# Autodesk Inventor assembly: Robot
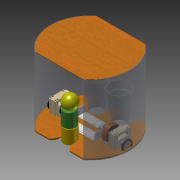
[picture p0: Inventor's stored thumbnail of the model, 180x180]
Saved by Autodesk Inventor 2014 SP1 (Build 180222100, 222)
## iProperties
Created: 2015-03-22
Part Number: Robot
Document SubType Name: Assembly
Designer: david
Mass: 1224.47 g
Surface Area: 3724.37 cm^2
Volume: 783.381 cm^3
Density: 1.56306 g/cm^3
Author: david
## Documents named in this file (19)
- C:\Users\asus\Documents\Autodesk\Projects\AUSBEEDone\Coupe2015\Robot.iam
- C:\Users\asus\Documents\Autodesk\Projects\AUSBEEDone\Components\EncoderBlock.iam
- C:\Users\asus\Documents\Autodesk\Projects\AUSBEEDone\Components\EncoderSupportOutside.ipt
- C:\Users\asus\Documents\Autodesk\Projects\AUSBEEDone\Components\Fasteners\ThreadedRod_M3_EncoderSupportInside.ipt
- C:\Users\asus\Documents\Autodesk\Projects\AUSBEEDone\Components\Fasteners\ThreadedRod_M3_EncoderSupportChassis.ipt
- C:\Users\asus\Documents\Autodesk\Projects\AUSBEEDone\Components\Fasteners\NylstopNut_M3.ipt
- C:\Users\asus\Documents\Autodesk\Projects\AUSBEEDone\Components\Fasteners\CompressionCoilSpring_5.5x35.ipt
- C:\Users\asus\Documents\Autodesk\Projects\AUSBEEDone\Components\Linking\Bracket.ipt
- C:\Users\asus\Documents\Autodesk\Projects\AUSBEEDone\Components\Linking\BracketUnfolded.ipt
- C:\Users\asus\Documents\Autodesk\Projects\AUSBEEDone\Components\Linking\BracketHalf.ipt
- C:\Users\asus\Documents\Autodesk\Projects\AUSBEEDone\Components\Motors\MotorBlockOneWheel.iam
- C:\Users\asus\Documents\Autodesk\Projects\AUSBEEDone\Coupe2015\ChassisRound.ipt
- C:\Users\asus\Documents\Autodesk\Projects\AUSBEEDone\Components\Motors\MotorBlockTwoWheels.iam
- C:\Users\asus\Documents\Autodesk\Projects\AUSBEEDone\Coupe2015\RoofRound.ipt
- C:\Users\asus\Documents\Autodesk\Projects\AUSBEEDone\Coupe2015\SideRound.ipt
- C:\Users\asus\Documents\Autodesk\Projects\AUSBEEDone\Coupe2015\PlayingElements\LightBulb_MaxSize.ipt
- C:\Users\asus\Documents\Autodesk\Projects\AUSBEEDone\Coupe2015\PlayingElements\StandGreen.ipt
- C:\Users\asus\Documents\Autodesk\Projects\AUSBEEDone\Coupe2015\PlayingElements\StandYellow.ipt
- C:\Users\asus\Documents\Autodesk\Projects\AUSBEEDone\Coupe2015\PlayingElements\PopcornCup.ipt
## Components (73 placed, 18 different names)
1. ChassisRound:1 — Mate:1, Mate:2, Cylindrical:25, Cylindrical:26, Mate:15, Mate:16, Mate:17, Mate:18, Mate:28, Mate:29, Mate:30, Mate:31, Mate:97, Mate:98, Angle:1, Mate:106, Mate:107, Angle:2, Mate:121, Mate:122, Mate:123, Mate:124, Mate:125, Mate:126, Mate:127
2. EncoderBlock:1 [sub-assembly] — Cylindrical:5, Cylindrical:6, Cylindrical:7, Cylindrical:8, Mate:7, Mate:8, Mate:9, Mate:10, Mate:44, Mate:45, Mate:46, Mate:47
3. EncoderBlock:2 [sub-assembly] — Cylindrical:9, Cylindrical:10, Cylindrical:11, Cylindrical:12, Mate:3, Mate:4, Mate:5, Mate:6, Flush:16, Mate:38, Mate:39, Mate:40, Tangent:1
4. MotorBlockOneWheel:1 [sub-assembly] — Mate:112, Mate:113, Mate:114
5. MotorBlockTwoWheels:1 [sub-assembly] — Mate:117, Mate:118, Mate:119, Mate:120
6. EncoderSupportOutside:1 — Cylindrical:1, Cylindrical:2, Cylindrical:3, Cylindrical:4, Mate:1, Cylindrical:21, Cylindrical:22, Cylindrical:23, Cylindrical:24, Flush:17
7. EncoderSupportOutside:2 — Mate:2, Cylindrical:13, Cylindrical:14, Cylindrical:15, Cylindrical:16, Cylindrical:29, Cylindrical:30, Cylindrical:31, Cylindrical:32, Mate:37
8. ThreadedRod_M3_EncoderSupportInside:1 — Cylindrical:3, Cylindrical:7, Mate:10, Mate:49, Mate:56, Flush:20
9. ThreadedRod_M3_EncoderSupportInside:2 — Cylindrical:1, Cylindrical:8, Mate:8, Mate:50, Mate:59, Flush:18
10. ThreadedRod_M3_EncoderSupportInside:3 — Cylindrical:4, Cylindrical:6, Mate:7, Mate:51, Mate:58, Flush:19
11. ThreadedRod_M3_EncoderSupportInside:4 — Cylindrical:2, Cylindrical:5, Mate:9, Mate:48, Mate:57, Flush:21
12. ThreadedRod_M3_EncoderSupportInside:5 — Cylindrical:9, Cylindrical:14, Mate:5, Mate:42, Mate:52, Flush:23
13. ThreadedRod_M3_EncoderSupportInside:6 — Cylindrical:10, Cylindrical:16, Mate:4, Mate:41, Mate:53, Flush:22
14. ThreadedRod_M3_EncoderSupportInside:7 — Cylindrical:12, Cylindrical:13, Mate:6, Mate:43, Mate:55, Flush:25
15. ThreadedRod_M3_EncoderSupportInside:8 — Cylindrical:11, Cylindrical:15, Mate:3, Mate:36, Mate:54, Flush:24
16. ThreadedRod_M3_EncoderSupportChassis:1 — Cylindrical:22, Mate:24, Flush:11, Mate:33, Flush:15, Mate:121
17. ThreadedRod_M3_EncoderSupportChassis:2 — Cylindrical:21, Mate:25, Flush:10, Mate:32, Flush:12
18. ThreadedRod_M3_EncoderSupportChassis:3 — Cylindrical:24, Mate:26, Flush:9, Flush:14, Mate:35, Mate:122
19. ThreadedRod_M3_EncoderSupportChassis:4 — Cylindrical:23, Mate:27, Flush:8, Mate:34, Flush:13
20. ThreadedRod_M3_EncoderSupportChassis:5 — Cylindrical:29, Mate:12, Flush:2, Mate:22, Flush:6
21. ThreadedRod_M3_EncoderSupportChassis:6 — Cylindrical:30, Mate:11, Flush:1, Mate:21, Flush:7
22. ThreadedRod_M3_EncoderSupportChassis:7 — Cylindrical:25, Cylindrical:32, Flush:3, Mate:13, Mate:19, Mate:23
23. ThreadedRod_M3_EncoderSupportChassis:8 — Cylindrical:26, Cylindrical:31, Mate:14, Flush:4, Mate:20, Flush:5
24. NylstopNut_M3:1 — Mate:14, Flush:4, Mate:16
25. NylstopNut_M3:2 — Flush:3, Mate:13, Mate:15
26. NylstopNut_M3:3 — Mate:11, Flush:1, Mate:17
27. NylstopNut_M3:4 — Mate:12, Flush:2, Mate:18
28. NylstopNut_M3:5 — Mate:20, Flush:5
29. NylstopNut_M3:6 — Mate:22, Flush:6
30. NylstopNut_M3:7 — Mate:21, Flush:7
31. NylstopNut_M3:8 — Mate:19, Mate:23
32. NylstopNut_M3:9 — Mate:27, Flush:8, Mate:31
33. NylstopNut_M3:10 — Mate:26, Flush:9, Mate:30
34. NylstopNut_M3:11 — Mate:25, Flush:10, Mate:29
35. NylstopNut_M3:12 — Mate:24, Flush:11, Mate:28
36. NylstopNut_M3:13 — Mate:33, Flush:15
37. NylstopNut_M3:14 — Mate:34, Flush:13
38. NylstopNut_M3:15 — Mate:32, Flush:12
39. NylstopNut_M3:16 — Flush:14, Mate:35
40. CompressionCoilSpring_5.5x35:1 — Mate:36, Flush:16, Mate:37
41. CompressionCoilSpring_5.5x35:2 — Mate:40, Mate:41
42. CompressionCoilSpring_5.5x35:3 — Mate:39, Mate:42
43. CompressionCoilSpring_5.5x35:4 — Mate:38, Mate:43
44. CompressionCoilSpring_5.5x35:5 — Mate:44, Mate:48, Flush:17
45. CompressionCoilSpring_5.5x35:6 — Mate:45, Mate:49
46. CompressionCoilSpring_5.5x35:7 — Mate:46, Mate:50
47. CompressionCoilSpring_5.5x35:8 — Mate:47, Mate:51
48. NylstopNut_M3:17 — Mate:57, Flush:21
49. NylstopNut_M3:18 — Mate:56, Flush:20
50. NylstopNut_M3:19 — Mate:59, Flush:18
51. NylstopNut_M3:20 — Mate:58, Flush:19
52. NylstopNut_M3:21 — Mate:52, Flush:23
53. NylstopNut_M3:22 — Mate:53, Flush:22
54. NylstopNut_M3:23 — Mate:55, Flush:25
55. NylstopNut_M3:24 — Mate:54, Flush:24
56. Bracket:1 — Mate:60, Mate:61, Mate:62, Mate:98, Mate:117, Mate:119
57. Bracket:2 — Mate:74, Mate:75, Mate:76, Mate:114
58. BracketUnfolded:1 — Mate:60, Mate:61, Mate:62, Mate:68, Mate:70, Mate:102
59. Bracket:3 — Mate:81, Mate:82, Mate:83, Mate:97, Mate:107, Mate:118, Mate:120
60. Bracket:4 — Mate:84, Mate:85, Mate:86, Mate:106, Mate:112, Mate:113
61. BracketUnfolded:4 — Mate:69, Mate:71, Mate:74, Mate:75, Mate:76, Mate:101
62. BracketHalf:1 — Mate:87, Mate:88, Mate:89, Mate:90, Mate:103
63. BracketHalf:2 — Mate:68, Mate:69, Mate:70, Mate:71, Mate:101, Mate:102
64. BracketUnfolded:5 — Mate:81, Mate:82, Mate:83, Mate:89, Mate:90, Mate:103
65. BracketUnfolded:6 — Mate:84, Mate:85, Mate:86, Mate:87, Mate:88
66. RoofRound:1 — Mate:128, Mate:129, Mate:131
67. SideRound:1 — Mate:125, Mate:126, Mate:127, Mate:128, Mate:129
68. SideRound:2 — Mate:123, Mate:124, Mate:131
69. LightBulb_MaxSize:1
70. StandGreen:1
71. StandYellow:1
72. PopcornCup:2
73. PopcornCup:4
## Relationships (157: Mate 103, CylindricalJoint 26, Flush 25, Angle 2, Tangent 1)
- Cylindrical:1: EncoderSupportOutside:1 ↔ ThreadedRod_M3_EncoderSupportInside:2
- Cylindrical:2: EncoderSupportOutside:1 ↔ ThreadedRod_M3_EncoderSupportInside:4
- Cylindrical:3: EncoderSupportOutside:1 ↔ ThreadedRod_M3_EncoderSupportInside:1
- Cylindrical:4: EncoderSupportOutside:1 ↔ ThreadedRod_M3_EncoderSupportInside:3
- Cylindrical:5: EncoderBlock:1 ↔ ThreadedRod_M3_EncoderSupportInside:4
- Mate:1: ChassisRound:1 ↔ EncoderSupportOutside:1
- Cylindrical:6: EncoderBlock:1 ↔ ThreadedRod_M3_EncoderSupportInside:3
- Cylindrical:7: EncoderBlock:1 ↔ ThreadedRod_M3_EncoderSupportInside:1
- Cylindrical:8: EncoderBlock:1 ↔ ThreadedRod_M3_EncoderSupportInside:2
- Mate:2: ChassisRound:1 ↔ EncoderSupportOutside:2
- Cylindrical:9: EncoderBlock:2 ↔ ThreadedRod_M3_EncoderSupportInside:5
- Cylindrical:10: EncoderBlock:2 ↔ ThreadedRod_M3_EncoderSupportInside:6
- Cylindrical:11: EncoderBlock:2 ↔ ThreadedRod_M3_EncoderSupportInside:8
- Cylindrical:12: EncoderBlock:2 ↔ ThreadedRod_M3_EncoderSupportInside:7
- Cylindrical:13: EncoderSupportOutside:2 ↔ ThreadedRod_M3_EncoderSupportInside:7
- Cylindrical:14: EncoderSupportOutside:2 ↔ ThreadedRod_M3_EncoderSupportInside:5
- Cylindrical:15: EncoderSupportOutside:2 ↔ ThreadedRod_M3_EncoderSupportInside:8
- Cylindrical:16: EncoderSupportOutside:2 ↔ ThreadedRod_M3_EncoderSupportInside:6
- Cylindrical:21: EncoderSupportOutside:1 ↔ ThreadedRod_M3_EncoderSupportChassis:2
- Cylindrical:22: EncoderSupportOutside:1 ↔ ThreadedRod_M3_EncoderSupportChassis:1
- Cylindrical:23: EncoderSupportOutside:1 ↔ ThreadedRod_M3_EncoderSupportChassis:4
- Cylindrical:24: EncoderSupportOutside:1 ↔ ThreadedRod_M3_EncoderSupportChassis:3
- Cylindrical:25: ChassisRound:1 ↔ ThreadedRod_M3_EncoderSupportChassis:7
- Cylindrical:26: ChassisRound:1 ↔ ThreadedRod_M3_EncoderSupportChassis:8
- Cylindrical:29: EncoderSupportOutside:2 ↔ ThreadedRod_M3_EncoderSupportChassis:5
- Cylindrical:30: EncoderSupportOutside:2 ↔ ThreadedRod_M3_EncoderSupportChassis:6
- Cylindrical:31: EncoderSupportOutside:2 ↔ ThreadedRod_M3_EncoderSupportChassis:8
- Cylindrical:32: EncoderSupportOutside:2 ↔ ThreadedRod_M3_EncoderSupportChassis:7
- Mate:3: EncoderBlock:2 ↔ ThreadedRod_M3_EncoderSupportInside:8
- Mate:4: EncoderBlock:2 ↔ ThreadedRod_M3_EncoderSupportInside:6
- Mate:5: EncoderBlock:2 ↔ ThreadedRod_M3_EncoderSupportInside:5
- Mate:6: EncoderBlock:2 ↔ ThreadedRod_M3_EncoderSupportInside:7
- Mate:7: EncoderBlock:1 ↔ ThreadedRod_M3_EncoderSupportInside:3
- Mate:8: EncoderBlock:1 ↔ ThreadedRod_M3_EncoderSupportInside:2
- Mate:9: EncoderBlock:1 ↔ ThreadedRod_M3_EncoderSupportInside:4
- Mate:10: EncoderBlock:1 ↔ ThreadedRod_M3_EncoderSupportInside:1
- Mate:11: ThreadedRod_M3_EncoderSupportChassis:6 ↔ NylstopNut_M3:3
- Flush:1: ThreadedRod_M3_EncoderSupportChassis:6 ↔ NylstopNut_M3:3
- Mate:12: ThreadedRod_M3_EncoderSupportChassis:5 ↔ NylstopNut_M3:4
- Flush:2: ThreadedRod_M3_EncoderSupportChassis:5 ↔ NylstopNut_M3:4
- Flush:3: ThreadedRod_M3_EncoderSupportChassis:7 ↔ NylstopNut_M3:2
- Mate:13: ThreadedRod_M3_EncoderSupportChassis:7 ↔ NylstopNut_M3:2
- Mate:14: ThreadedRod_M3_EncoderSupportChassis:8 ↔ NylstopNut_M3:1
- Flush:4: ThreadedRod_M3_EncoderSupportChassis:8 ↔ NylstopNut_M3:1
- Mate:15: ChassisRound:1 ↔ NylstopNut_M3:2
- Mate:16: ChassisRound:1 ↔ NylstopNut_M3:1
- Mate:17: ChassisRound:1 ↔ NylstopNut_M3:3
- Mate:18: ChassisRound:1 ↔ NylstopNut_M3:4
- Mate:19: ThreadedRod_M3_EncoderSupportChassis:7 ↔ NylstopNut_M3:8
- Mate:20: ThreadedRod_M3_EncoderSupportChassis:8 ↔ NylstopNut_M3:5
- Mate:21: ThreadedRod_M3_EncoderSupportChassis:6 ↔ NylstopNut_M3:7
- Mate:22: ThreadedRod_M3_EncoderSupportChassis:5 ↔ NylstopNut_M3:6
- Mate:23: ThreadedRod_M3_EncoderSupportChassis:7 ↔ NylstopNut_M3:8
- Flush:5: ThreadedRod_M3_EncoderSupportChassis:8 ↔ NylstopNut_M3:5
- Flush:6: ThreadedRod_M3_EncoderSupportChassis:5 ↔ NylstopNut_M3:6
- Flush:7: ThreadedRod_M3_EncoderSupportChassis:6 ↔ NylstopNut_M3:7
- Mate:24: ThreadedRod_M3_EncoderSupportChassis:1 ↔ NylstopNut_M3:12
- Mate:25: ThreadedRod_M3_EncoderSupportChassis:2 ↔ NylstopNut_M3:11
- Mate:26: ThreadedRod_M3_EncoderSupportChassis:3 ↔ NylstopNut_M3:10
- Mate:27: ThreadedRod_M3_EncoderSupportChassis:4 ↔ NylstopNut_M3:9
- Flush:8: ThreadedRod_M3_EncoderSupportChassis:4 ↔ NylstopNut_M3:9
- Flush:9: ThreadedRod_M3_EncoderSupportChassis:3 ↔ NylstopNut_M3:10
- Flush:10: ThreadedRod_M3_EncoderSupportChassis:2 ↔ NylstopNut_M3:11
- Flush:11: ThreadedRod_M3_EncoderSupportChassis:1 ↔ NylstopNut_M3:12
- Mate:28: ChassisRound:1 ↔ NylstopNut_M3:12
- Mate:29: ChassisRound:1 ↔ NylstopNut_M3:11
- Mate:30: ChassisRound:1 ↔ NylstopNut_M3:10
- Mate:31: ChassisRound:1 ↔ NylstopNut_M3:9
- Mate:32: ThreadedRod_M3_EncoderSupportChassis:2 ↔ NylstopNut_M3:15
- Flush:12: ThreadedRod_M3_EncoderSupportChassis:2 ↔ NylstopNut_M3:15
- Mate:33: ThreadedRod_M3_EncoderSupportChassis:1 ↔ NylstopNut_M3:13
- Mate:34: ThreadedRod_M3_EncoderSupportChassis:4 ↔ NylstopNut_M3:14
- Flush:13: ThreadedRod_M3_EncoderSupportChassis:4 ↔ NylstopNut_M3:14
- Flush:14: ThreadedRod_M3_EncoderSupportChassis:3 ↔ NylstopNut_M3:16
- Flush:15: ThreadedRod_M3_EncoderSupportChassis:1 ↔ NylstopNut_M3:13
- Mate:35: ThreadedRod_M3_EncoderSupportChassis:3 ↔ NylstopNut_M3:16
- Mate:36: ThreadedRod_M3_EncoderSupportInside:8 ↔ CompressionCoilSpring_5.5x35:1
- Flush:16: EncoderBlock:2 ↔ CompressionCoilSpring_5.5x35:1
- Mate:37: EncoderSupportOutside:2 ↔ CompressionCoilSpring_5.5x35:1
- Mate:38: EncoderBlock:2 ↔ CompressionCoilSpring_5.5x35:4
- Mate:39: EncoderBlock:2 ↔ CompressionCoilSpring_5.5x35:3
- Mate:40: EncoderBlock:2 ↔ CompressionCoilSpring_5.5x35:2
- Mate:41: ThreadedRod_M3_EncoderSupportInside:6 ↔ CompressionCoilSpring_5.5x35:2
- Mate:42: ThreadedRod_M3_EncoderSupportInside:5 ↔ CompressionCoilSpring_5.5x35:3
- Mate:43: ThreadedRod_M3_EncoderSupportInside:7 ↔ CompressionCoilSpring_5.5x35:4
- Mate:44: EncoderBlock:1 ↔ CompressionCoilSpring_5.5x35:5
- Mate:45: EncoderBlock:1 ↔ CompressionCoilSpring_5.5x35:6
- Mate:46: EncoderBlock:1 ↔ CompressionCoilSpring_5.5x35:7
- Mate:47: EncoderBlock:1 ↔ CompressionCoilSpring_5.5x35:8
- Mate:48: ThreadedRod_M3_EncoderSupportInside:4 ↔ CompressionCoilSpring_5.5x35:5
- Mate:49: ThreadedRod_M3_EncoderSupportInside:1 ↔ CompressionCoilSpring_5.5x35:6
- Mate:50: ThreadedRod_M3_EncoderSupportInside:2 ↔ CompressionCoilSpring_5.5x35:7
- Mate:51: ThreadedRod_M3_EncoderSupportInside:3 ↔ CompressionCoilSpring_5.5x35:8
- Flush:17: EncoderSupportOutside:1 ↔ CompressionCoilSpring_5.5x35:5
- Mate:52: ThreadedRod_M3_EncoderSupportInside:5 ↔ NylstopNut_M3:21
- Mate:53: ThreadedRod_M3_EncoderSupportInside:6 ↔ NylstopNut_M3:22
- Mate:54: ThreadedRod_M3_EncoderSupportInside:8 ↔ NylstopNut_M3:24
- Mate:55: ThreadedRod_M3_EncoderSupportInside:7 ↔ NylstopNut_M3:23
- Mate:56: ThreadedRod_M3_EncoderSupportInside:1 ↔ NylstopNut_M3:18
- Mate:57: ThreadedRod_M3_EncoderSupportInside:4 ↔ NylstopNut_M3:17
- Mate:58: ThreadedRod_M3_EncoderSupportInside:3 ↔ NylstopNut_M3:20
- Mate:59: ThreadedRod_M3_EncoderSupportInside:2 ↔ NylstopNut_M3:19
- Flush:18: ThreadedRod_M3_EncoderSupportInside:2 ↔ NylstopNut_M3:19
- Flush:19: ThreadedRod_M3_EncoderSupportInside:3 ↔ NylstopNut_M3:20
- Flush:20: ThreadedRod_M3_EncoderSupportInside:1 ↔ NylstopNut_M3:18
- Flush:21: ThreadedRod_M3_EncoderSupportInside:4 ↔ NylstopNut_M3:17
- Flush:22: ThreadedRod_M3_EncoderSupportInside:6 ↔ NylstopNut_M3:22
- Flush:23: ThreadedRod_M3_EncoderSupportInside:5 ↔ NylstopNut_M3:21
- Flush:24: ThreadedRod_M3_EncoderSupportInside:8 ↔ NylstopNut_M3:24
- Flush:25: ThreadedRod_M3_EncoderSupportInside:7 ↔ NylstopNut_M3:23
- Mate:60: Bracket:1 ↔ BracketUnfolded:1
- Mate:61: Bracket:1 ↔ BracketUnfolded:1
- Mate:62: Bracket:1 ↔ BracketUnfolded:1
- Mate:68: BracketUnfolded:1 ↔ BracketHalf:2
- Mate:69: BracketUnfolded:4 ↔ BracketHalf:2
- Mate:70: BracketUnfolded:1 ↔ BracketHalf:2
- Mate:71: BracketUnfolded:4 ↔ BracketHalf:2
- Mate:74: Bracket:2 ↔ BracketUnfolded:4
- Mate:75: Bracket:2 ↔ BracketUnfolded:4
- Mate:76: Bracket:2 ↔ BracketUnfolded:4
- Mate:81: Bracket:3 ↔ BracketUnfolded:5
- Mate:82: Bracket:3 ↔ BracketUnfolded:5
- Mate:83: Bracket:3 ↔ BracketUnfolded:5
- Mate:84: Bracket:4 ↔ BracketUnfolded:6
- Mate:85: Bracket:4 ↔ BracketUnfolded:6
- Mate:86: Bracket:4 ↔ BracketUnfolded:6
- Mate:87: BracketHalf:1 ↔ BracketUnfolded:6
- Mate:88: BracketHalf:1 ↔ BracketUnfolded:6
- Mate:89: BracketHalf:1 ↔ BracketUnfolded:5
- Mate:90: BracketHalf:1 ↔ BracketUnfolded:5
- Mate:97: ChassisRound:1 ↔ Bracket:3
- Mate:98: ChassisRound:1 ↔ Bracket:1
- Angle:1 (0 deg): ChassisRound:1
- Tangent:1: EncoderBlock:2
- Mate:101: BracketUnfolded:4 ↔ BracketHalf:2
- Mate:102: BracketUnfolded:1 ↔ BracketHalf:2
- Mate:103: BracketHalf:1 ↔ BracketUnfolded:5
- Mate:106: ChassisRound:1 ↔ Bracket:4
- Mate:107: ChassisRound:1 ↔ Bracket:3
- Angle:2 (0 deg): ChassisRound:1
- Mate:112: MotorBlockOneWheel:1 ↔ Bracket:4
- Mate:113: MotorBlockOneWheel:1 ↔ Bracket:4
- Mate:114: MotorBlockOneWheel:1 ↔ Bracket:2
- Mate:117: MotorBlockTwoWheels:1 ↔ Bracket:1
- Mate:118: MotorBlockTwoWheels:1 ↔ Bracket:3
- Mate:119: MotorBlockTwoWheels:1 ↔ Bracket:1
- Mate:120: MotorBlockTwoWheels:1 ↔ Bracket:3
- Mate:121: ChassisRound:1 ↔ ThreadedRod_M3_EncoderSupportChassis:1
- Mate:122: ChassisRound:1 ↔ ThreadedRod_M3_EncoderSupportChassis:3
- Mate:123: ChassisRound:1 ↔ SideRound:2
- Mate:124: ChassisRound:1 ↔ SideRound:2
- Mate:125: ChassisRound:1 ↔ SideRound:1
- Mate:126: ChassisRound:1 ↔ SideRound:1
- Mate:127: ChassisRound:1 ↔ SideRound:1
- Mate:128: RoofRound:1 ↔ SideRound:1
- Mate:129: RoofRound:1 ↔ SideRound:1
- Mate:131: RoofRound:1 ↔ SideRound:2
## Named parameters: EncoderBlock_BodyToWheel_Distance = 24.5 mm
